# Autodesk Inventor assembly: arm_shift_1
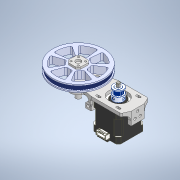
[picture p0: Inventor's stored thumbnail of the model, 180x180]
Saved by Autodesk Inventor 2020 (Build 240168000, 168)
## iProperties
Created: 2020-01-18
Part Number: arm_shift_1
Document SubType Name: Assembly
Designer: psrobotics
Author: psrobotics
## Documents named in this file (8)
- F:\projects-3\delta_arm\hardware\arm_shift_1.iam
- F:\projects-3\delta_arm\hardware\Nema17 Stepper Motor.ipt
- F:\projects-3\delta_arm\hardware\source\gt2-timing-pulley-configurable-16t-20t-b3-b8-w3-w6-w10-1.snapshot.1\Step files\GT2 Timing Pulley, Configurable, 20T W6 B5.iam
- F:\projects-3\delta_arm\hardware\motor_holder_1.ipt
- F:\projects-3\delta_arm\hardware\120teeth gt2 pulley.ipt
- F:\projects-3\delta_arm\hardware\pin_8_45.ipt
- F:\projects-3\delta_arm\hardware\pin_holder_1.ipt
- F:\projects-3\delta_arm\hardware\bearing_8_16_5.ipt
## Components (8 placed, 7 different names)
1. Nema17 Stepper Motor:1 — Insert:1, Flush:1, Flush:2, Mate:1
2. GT2 Timing Pulley, Configurable, 20T W6 B5:1 [sub-assembly] — Insert:1
3. motor_holder_1:1 — Flush:1, Flush:2, Mate:1, Insert:2, Insert:6, Insert:7
4. 120teeth gt2 pulley:1 — Insert:2, Insert:3, Flush:3, Insert:4, Insert:5
5. pin_8_45:1 — Insert:3
6. pin_holder_1:1 — Flush:3, Insert:4, Insert:5
7. bearing_8_16_5:1 — Insert:6
8. bearing_8_16_5:2 — Insert:7
## Relationships (11: Insert 7, Flush 3, Mate 1)
- Insert:1: Nema17 Stepper Motor:1 ↔ GT2 Timing Pulley, Configurable, 20T W6 B5:1
- Flush:1: Nema17 Stepper Motor:1 ↔ motor_holder_1:1
- Flush:2: Nema17 Stepper Motor:1 ↔ motor_holder_1:1
- Mate:1 (4 mm): Nema17 Stepper Motor:1 ↔ motor_holder_1:1
- Insert:2: motor_holder_1:1 ↔ 120teeth gt2 pulley:1
- Insert:3: 120teeth gt2 pulley:1 ↔ pin_8_45:1
- Flush:3: 120teeth gt2 pulley:1 ↔ pin_holder_1:1
- Insert:4: 120teeth gt2 pulley:1 ↔ pin_holder_1:1
- Insert:5: 120teeth gt2 pulley:1 ↔ pin_holder_1:1
- Insert:6: motor_holder_1:1 ↔ bearing_8_16_5:1
- Insert:7: motor_holder_1:1 ↔ bearing_8_16_5:2
